# Autodesk Inventor assembly: movementfinal
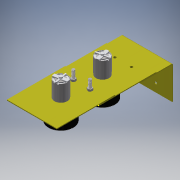
[picture p0: Inventor's stored thumbnail of the model, 180x180]
Saved by Autodesk Inventor 2019 (Build 230136000, 136)
## iProperties
Created: 2020-02-14
Part Number: movementfinal
Document SubType Name: Assembly
Designer: Dell
Author: Dell
## Documents named in this file (8)
- C:\Users\Dell\Documents\movementfinal.iam
- C:\Users\Dell\Documents\movement.ipt
- C:\Users\Dell\Documents\nut2.ipt
- C:\Users\Dell\Documents\bolt.ipt
- C:\Users\Dell\Documents\clamp.ipt
- C:\Users\Dell\Documents\motordc2.ipt
- C:\Users\Dell\Documents\movement2.ipt
- C:\Users\Dell\Documents\carromwheel2.ipt
## Components (11 placed, 7 different names)
1. movement:1 — Rotational:4, Rotational:5, Rigid:3, Rigid:4, Rotational:9
2. motordc2:1 — Rotational:4, Rigid:5
3. movement2:1 — Rotational:5, Rotational:6, Rotational:7, Rotational:8
4. bolt:3 — Rigid:4
5. bolt:4 — Rigid:3
6. nut2:3 — Rotational:6
7. nut2:4 — Rotational:7
8. motordc2:2 — Rotational:8, Rigid:6
9. carromwheel2:1 — Rigid:6
10. carromwheel2:2 — Rigid:5
11. clamp:1 — Rotational:9
## Relationships (10: RevoluteJoint 6, WeldJoint 4)
- Rotational:4 [RevoluteJoint]: movement:1 ↔ motordc2:1
- Rotational:5 [RevoluteJoint]: movement:1 ↔ movement2:1
- Rigid:3 [WeldJoint]: movement:1 ↔ bolt:4
- Rigid:4 [WeldJoint]: movement:1 ↔ bolt:3
- Rotational:6 [RevoluteJoint]: movement2:1 ↔ nut2:3
- Rotational:7 [RevoluteJoint]: movement2:1 ↔ nut2:4
- Rotational:8 [RevoluteJoint]: movement2:1 ↔ motordc2:2
- Rigid:5 [WeldJoint]: motordc2:1 ↔ carromwheel2:2
- Rigid:6 [WeldJoint]: motordc2:2 ↔ carromwheel2:1
- Rotational:9 [RevoluteJoint]: movement:1 ↔ clamp:1
